# Autodesk Inventor assembly: terminal
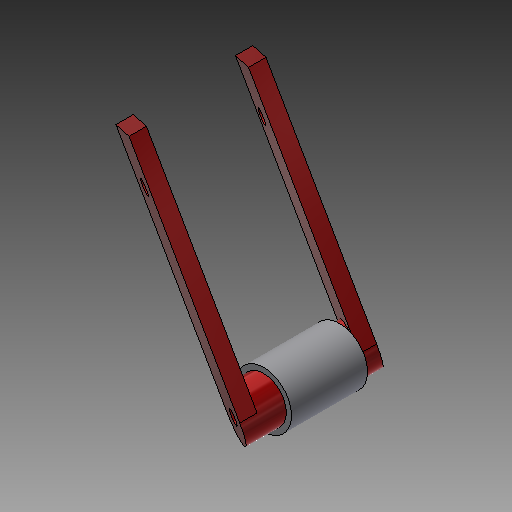
[picture p0: Inventor's stored thumbnail of the model, 512x512]
Saved by Autodesk Inventor 2018 (Build 220112000, 112)
## iProperties
Created: 2017-06-03
Part Number: terminal
Document SubType Name: Assembly
Designer: AYUSH SHUKLA
Author: AYUSH SHUKLA
## Documents named in this file (9)
- C:\Study\BTP2\Robomuse Inventor CAD\Terminal\terminal_complete.iam
- C:\Study\BTP2\Robomuse Inventor CAD\Terminal\terminal.ipt
- C:\Study\BTP2\Robomuse Inventor CAD\Terminal\terminal_mount.ipt
- C:\Study\BTP2\Robomuse Inventor CAD\terminal\AIP\FEA\c61dem4w0.fins
- C:\Study\BTP2\Robomuse Inventor CAD\terminal\AIP\FEA\c61dem4w0.fsat
- C:\Study\BTP2\Robomuse Inventor CAD\terminal\AIP\FEA\c61dem4w0.ftes
- C:\Study\BTP2\Robomuse Inventor CAD\terminal\AIP\FEA\c61dem4w0.fwiz
- C:\Study\BTP2\Robomuse Inventor CAD\terminal\AIP\FEA\c61dem4xs.fmsh
- C:\Study\BTP2\Robomuse Inventor CAD\terminal\AIP\FEA\c61dem4xt.fres
## Components (3 placed, 2 different names)
1. terminal:1 — Mate:1, Mate:2, Mate:4
2. terminal_mount:1 — Mate:1, Angle:1, Mate:3
3. terminal_mount:2 — Angle:1, Mate:2, Mate:3, Mate:4
## Relationships (5: Mate 4, Angle 1)
- Mate:1: terminal:1 ↔ terminal_mount:1
- Angle:1 (0 deg): terminal_mount:1 ↔ terminal_mount:2
- Mate:2: terminal:1 ↔ terminal_mount:2
- Mate:3 (29.3294 mm): terminal_mount:1 ↔ terminal_mount:2
- Mate:4: terminal:1 ↔ terminal_mount:2
## Named parameters: sa_0 = 9832.79, sa_1 = 1821.04, sa_2 = 2.02e-11
note: some values were not read from the file. Shown as the stored number, unit unknown: "sa_0", "sa_1", "sa_2".
